# Autodesk Inventor assembly: Assembly1
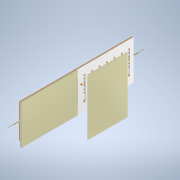
[picture p0: Inventor's stored thumbnail of the model, 180x180]
Saved by Autodesk Inventor 2020 (Build 240168000, 168)
## iProperties
Created: 2021-01-27
Part Number: Assembly1
Document SubType Name: Assembly
Designer: abij996
Author: abij996
## Documents named in this file (4)
- \\files.auckland.ac.nz\myhome\Documents\GitHub\2020-srw-rc-car\CoilDesign\CAD Track\Assembly1.iam
- \\files.auckland.ac.nz\myhome\Documents\GitHub\2020-srw-rc-car\CoilDesign\CAD Track\Wire Cad Model\primary_coil_0R2.ipt
- \\files.auckland.ac.nz\myhome\Documents\GitHub\2020-srw-rc-car\CoilDesign\CAD Track\Ferrite Layer\2 sections\ferrite_section.ipt
- \\files.auckland.ac.nz\myhome\Documents\GitHub\2020-srw-rc-car\CoilDesign\CAD Track\Top Layer\TopCoverLayer.ipt
## Components (7 placed, 3 different names)
1. primary_coil_0R2:1 — Mate:2, Flush:2, Flush:3, Mate:3, Mate:4, Flush:6, Flush:7, Mate:5
2. ferrite_section:1 — Mate:1, Flush:1, Mate:2, Flush:2, Flush:3
3. ferrite_section:2 — Mate:1, Flush:1, Mate:3, Flush:4, Flush:5
4. TopCoverLayer:1 — Flush:4, Flush:5
5. TopCoverLayer:2 — Mate:4, Flush:6, Flush:7, Flush:8
6. TopCoverLayer:3 — Mate:5, Flush:8
7. TopCoverLayer:4
## Relationships (13: Flush 8, Mate 5)
- Mate:1: ferrite_section:1 ↔ ferrite_section:2
- Flush:1: ferrite_section:1 ↔ ferrite_section:2
- Mate:2: primary_coil_0R2:1 ↔ ferrite_section:1
- Flush:2: primary_coil_0R2:1 ↔ ferrite_section:1
- Flush:3: primary_coil_0R2:1 ↔ ferrite_section:1
- Mate:3: primary_coil_0R2:1 ↔ ferrite_section:2
- Flush:4: ferrite_section:2 ↔ TopCoverLayer:1
- Flush:5: ferrite_section:2 ↔ TopCoverLayer:1
- Mate:4: primary_coil_0R2:1 ↔ TopCoverLayer:2
- Flush:6: primary_coil_0R2:1 ↔ TopCoverLayer:2
- Flush:7: primary_coil_0R2:1 ↔ TopCoverLayer:2
- Mate:5: primary_coil_0R2:1 ↔ TopCoverLayer:3
- Flush:8: TopCoverLayer:2 ↔ TopCoverLayer:3
